# Autodesk Inventor assembly: Perna_Dir_Montada_v1
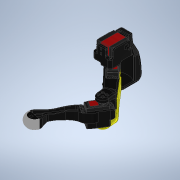
[picture p0: Inventor's stored thumbnail of the model, 180x180]
Saved by Autodesk Inventor 2020 (Build 240168000, 168)
## iProperties
Created: 2021-05-14
Part Number: Perna_Dir_Montada_v1
Document SubType Name: Assembly
Designer: JCarlos
Author: JCarlos
## Documents named in this file (10)
- C:\Users\candu\Google Drive\Doutorado_UTFPR\Projeto_1_SpotMicro\Projeto_3D\Robo_Montado_v3\Perna_Dir_Montada_v3.iam
- C:\Users\candu\Google Drive\Doutorado_UTFPR\Projeto_1_SpotMicro\Projeto_3D\Robo_Montado_v3\Ante_Braço_Dir.ipt
- C:\Users\candu\Google Drive\Doutorado_UTFPR\Projeto_1_SpotMicro\Projeto_3D\Robo_Montado_v3\Braço_Dir.ipt
- C:\Users\candu\Google Drive\Doutorado_UTFPR\Projeto_1_SpotMicro\Projeto_3D\Perna_Dir_Montada_v1\Design Accelerator\Rolamento1.iam
- C:\Users\candu\Google Drive\Doutorado_UTFPR\Projeto_1_SpotMicro\Projeto_3D\Robo_Montado_v3\foot.ipt
- C:\Users\candu\Google Drive\Doutorado_UTFPR\Projeto_1_SpotMicro\Projeto_3D\Robo_Montado_v3\Cover_Braço_Dir_v3.ipt
- C:\Users\candu\Google Drive\Doutorado_UTFPR\Projeto_1_SpotMicro\Projeto_3D\Robo_Montado_v3\LF20MG\Circle Rudder.ipt
- C:\Users\candu\Google Drive\Doutorado_UTFPR\Projeto_1_SpotMicro\Projeto_3D\Robo_Montado_v3\LF20MG\LF20MG.ipt
- C:\Users\candu\Google Drive\Doutorado_UTFPR\Projeto_1_SpotMicro\Projeto_3D\Robo_Montado_v3\Rótula_FrDir_TrEsq_v3.ipt
- C:\Users\candu\Google Drive\Doutorado_UTFPR\Projeto_1_SpotMicro\Projeto_3D\Robo_Montado_v3\Ombrera_Dir.ipt
## Components (11 placed, 9 different names)
1. Ante_Braço_Dir:1 — Coincidência:10, Coincidência:11, Coincidência:22, Coincidência:23, Coincidência:24, Coincidência:25
2. Cover_Braço_Dir_v3:1 — Coincidência:39, Coincidência:40
3. Braço_Dir:1 — Coincidência:3, Alinhamento:3, Coincidência:15, Coincidência:16, Coincidência:17, Coincidência:18, Coincidência:19, Tangente:1, Coincidência:28
4. Rolamento:1 [sub-assembly] — Coincidência:3
5. LF20MG:3 — Coincidência:17, Coincidência:18, Coincidência:19, Coincidência:20, Coincidência:21
6. LF20MG:4 — Coincidência:23, Coincidência:24, Coincidência:25, Coincidência:26, Coincidência:27
7. Circle Rudder:1 — Coincidência:10, Coincidência:11, Coincidência:20, Coincidência:21, Coincidência:22
8. foot:1 — Alinhamento:3, Coincidência:15, Coincidência:16
9. Rótula_FrDir_TrEsq_v3:1 — Coincidência:26, Coincidência:27, Ângulo:1, Ângulo:2, Coincidência:32, Coincidência:33, Coincidência:34, Coincidência:35
10. Ombrera_Dir:1 — Coincidência:36, Coincidência:37, Coincidência:38
11. LF20MG:5 — Coincidência:33, Coincidência:34, Coincidência:35, Coincidência:36, Coincidência:37, Coincidência:38
## Relationships (37: Mate 31, Flush 3, Angle 2, Tangent 1)
- [Mate]: Ante_Braço_Dir:1 ↔ Cover_Braço_Dir_v3:1
- [Flush]: Ante_Braço_Dir:1 ↔ Cover_Braço_Dir_v3:1
- [Mate]: Cover_Braço_Dir_v3:1 ↔ Rolamento:1
- [Flush]: Cover_Braço_Dir_v3:1 ↔ Rolamento:1
- Coincidência:3 [Mate]: Braço_Dir:1 ↔ Rolamento:1
- Coincidência:10 [Mate]: Ante_Braço_Dir:1 ↔ Circle Rudder:1
- Coincidência:11 [Mate]: Ante_Braço_Dir:1 ↔ Circle Rudder:1
- [Mate] (1 mm): Cover_Braço_Dir_v3:1 ↔ Braço_Dir:1
- [Mate]: Ante_Braço_Dir:1 ↔ Cover_Braço_Dir_v3:1
- Alinhamento:3 [Flush]: Braço_Dir:1 ↔ foot:1
- Coincidência:15 [Mate]: Braço_Dir:1 ↔ foot:1
- Coincidência:16 [Mate]: Braço_Dir:1 ↔ foot:1
- Coincidência:17 [Mate]: Braço_Dir:1 ↔ LF20MG:3
- Coincidência:18 [Mate]: Braço_Dir:1 ↔ LF20MG:3
- Coincidência:19 [Mate]: Braço_Dir:1 ↔ LF20MG:3
- Coincidência:20 [Mate]: LF20MG:3 ↔ Circle Rudder:1
- Coincidência:21 [Mate] (-46 mm): LF20MG:3 ↔ Circle Rudder:1
- Coincidência:22 [Mate]: Ante_Braço_Dir:1 ↔ Circle Rudder:1
- Coincidência:23 [Mate]: Ante_Braço_Dir:1 ↔ LF20MG:4
- Coincidência:24 [Mate]: Ante_Braço_Dir:1 ↔ LF20MG:4
- Coincidência:25 [Mate]: Ante_Braço_Dir:1 ↔ LF20MG:4
- Coincidência:26 [Mate]: LF20MG:4 ↔ Rótula_FrDir_TrEsq_v3:1
- Coincidência:27 [Mate] (3 mm): LF20MG:4 ↔ Rótula_FrDir_TrEsq_v3:1
- Ângulo:1 [Angle] (90 deg): Rótula_FrDir_TrEsq_v3:1
- Tangente:1: Braço_Dir:1
- Coincidência:28 [Mate]: Braço_Dir:1
- Coincidência:29 [Mate]
- Ângulo:2 [Angle] (90 deg): Rótula_FrDir_TrEsq_v3:1
- Coincidência:32 [Mate]: Rótula_FrDir_TrEsq_v3:1
- Coincidência:33 [Mate]: Rótula_FrDir_TrEsq_v3:1 ↔ LF20MG:5
- Coincidência:34 [Mate]: Rótula_FrDir_TrEsq_v3:1 ↔ LF20MG:5
- Coincidência:35 [Mate]: Rótula_FrDir_TrEsq_v3:1 ↔ LF20MG:5
- Coincidência:36 [Mate]: Ombrera_Dir:1 ↔ LF20MG:5
- Coincidência:37 [Mate]: Ombrera_Dir:1 ↔ LF20MG:5
- Coincidência:38 [Mate] (0.5 mm): Ombrera_Dir:1 ↔ LF20MG:5
- Coincidência:39 [Mate]: Cover_Braço_Dir_v3:1
- Coincidência:40 [Mate] (200 mm): Cover_Braço_Dir_v3:1
